# Autodesk Inventor assembly: Tuner
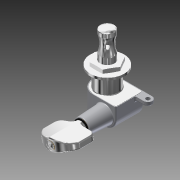
[picture p0: Inventor's stored thumbnail of the model, 180x180]
Saved by Autodesk Inventor 2014 (Build 180170000, 170)
## iProperties
Shininess: 3
Length Units: 11272
Angle Units: 11279
Time Units: 11290
Mass Units: 11286
Length Display Precision: 3
Angle Display Precision: 2
Compacted: True
Company: Autodesk, Inc.
Created: 2001-07-11
Part Number: Tuner
Document SubType Name: Assembly
Designer: Autodesk, Inc.
Mass: 52.3344 g
Surface Area: 86.6261 cm^2
Volume: 7.13657 cm^3
Density: 7.33327 g/cm^3
Density: 0.0
Volumn: 0.0
Area: 0.0
PropertySet Name: Model Information
Control State: 0
Master: False
Checked Out: False
Author: Autodesk, Inc.
## Documents named in this file (12)
- C:\Samples\Models\Assemblies\Tuner\Tuner.iam
- C:\Samples\Models\Assemblies\Tuner\Tuner Components\large cap.ipt
- C:\Samples\Models\Assemblies\Tuner\Tuner Components\small cap.ipt
- C:\Samples\Models\Assemblies\Tuner\Tuner Components\casting2.ipt
- C:\Samples\Models\Assemblies\Tuner\Tuner Components\shaft.ipt
- C:\Samples\Models\Assemblies\Tuner\Tuner Components\thrust washer.ipt
- C:\Samples\Models\Assemblies\Tuner\Tuner Components\button.ipt
- C:\Samples\Models\Assemblies\Tuner\Tuner Components\screw.ipt
- C:\Samples\Models\Assemblies\Tuner\Tuner Components\postcap.ipt
- C:\Samples\Models\Assemblies\Tuner\Tuner Components\hex sleeve.ipt
- C:\Samples\Models\Assemblies\Tuner\Tuner Components\trim washer.ipt
- C:\Samples\Models\Assemblies\Tuner\Tuner Components\string post.ipt
## Components (11 placed, 11 different names)
1. casting2:1 — Flush:1, Mate:1, Flush:2, Mate:2, Mate:3, Mate:11, Mate:12, Mate:13, Angle:1
2. large cap:1 — Flush:1, Mate:1, Mate:18
3. small cap:1 — Flush:2, Mate:2, Mate:4
4. shaft:1 — Mate:3, Mate:4, Mate:5, Mate:6, Mate:7, Mate:9, Mate:10
5. thrust washer:1 — Mate:5, Mate:6, Mate:8
6. button:1 — Mate:7, Mate:8, Angle:1, Rotation:1
7. screw:1 — Mate:9, Mate:10
8. postcap:1 — Mate:11, Mate:12, Mate:13, Mate:14, Mate:15, Mate:16
9. hex sleeve:1 — Mate:16, Mate:17, Mate:19
10. trim washer:1 — Mate:14, Mate:15, Mate:17
11. string post:1 — Mate:18, Rotation:1, Mate:19
## Relationships (23: Mate 19, Flush 2, Angle 1, RelateRotation 1)
- Flush:1: casting2:1 ↔ large cap:1
- Mate:1: casting2:1 ↔ large cap:1
- Flush:2: casting2:1 ↔ small cap:1
- Mate:2: casting2:1 ↔ small cap:1
- Mate:3: casting2:1 ↔ shaft:1
- Mate:4: small cap:1 ↔ shaft:1
- Mate:5: shaft:1 ↔ thrust washer:1
- Mate:6: shaft:1 ↔ thrust washer:1
- Mate:7: shaft:1 ↔ button:1
- Mate:8: thrust washer:1 ↔ button:1
- Mate:9: shaft:1 ↔ screw:1
- Mate:10 (0.508 mm): shaft:1 ↔ screw:1
- Mate:11: casting2:1 ↔ postcap:1
- Mate:12: casting2:1 ↔ postcap:1
- Mate:13: casting2:1 ↔ postcap:1
- Mate:14: postcap:1 ↔ trim washer:1
- Mate:15: postcap:1 ↔ trim washer:1
- Mate:16: postcap:1 ↔ hex sleeve:1
- Mate:17: hex sleeve:1 ↔ trim washer:1
- Mate:18: large cap:1 ↔ string post:1
- Angle:1 (0 deg): casting2:1 ↔ button:1
- Rotation:1 [RelateRotation] (0.0625 ul): button:1 ↔ string post:1
- Mate:19: hex sleeve:1 ↔ string post:1
